# Autodesk Inventor assembly: ASSEMBLY_Visual_inspection_tray
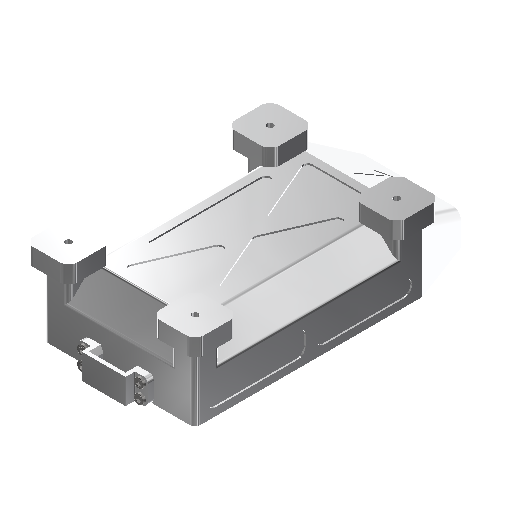
[picture p0: Inventor's stored thumbnail of the model, 512x512]
Saved by Autodesk Inventor 2025 (Build 290162010, 162A)
## iProperties
Created: 2018-09-18
Part Number: ASSEMBLY_Visual_inspection_tray
Document SubType Name: Assembly
Designer: Andrzej
Mass: 50.3843 g
Surface Area: 208.171 cm^2
Volume: 18.5637 cm^3
Density: 2.71413 g/cm^3
Author: Andrzej
## Documents named in this file (5)
- D:\_ANDRZEJ_LACZEWSKI\_OTHER\MECH - My entry for the NASA Lunar Sampling System Design Challenge\MCAD\1_REV1\ASSEMBLY_MAIN_REVA\ASSEMBLY_Visual_inspection_tray.iam
- D:\_ANDRZEJ_LACZEWSKI\_OTHER\MECH - My entry for the NASA Lunar Sampling System Design Challenge\MCAD\1_REV1\ASSEMBLY_MAIN_REVA\CNCM_ALU_Visual_inspection_tray.ipt
- D:\_ANDRZEJ_LACZEWSKI\_OTHER\MECH - My entry for the NASA Lunar Sampling System Design Challenge\MCAD\1_REV1\ASSEMBLY_MAIN_REVA\CNCM_ALU_Visual_inspection_tray_leg_holder.ipt
- D:\_ANDRZEJ_LACZEWSKI\_OTHER\MECH - My entry for the NASA Lunar Sampling System Design Challenge\MCAD\1_REV1\ASSEMBLY_MAIN_REVA\CNCM_ALU_Visial_inspection_tray_bucket_mount.ipt
- D:\_ANDRZEJ_LACZEWSKI\_OTHER\MECH - My entry for the NASA Lunar Sampling System Design Challenge\MCAD\1_REV1\ASSEMBLY_MAIN_REVA\CNCT_STEEL_M1,6x3,5_Screw.ipt
## Components (10 placed, 4 different names)
1. CNCM_ALU_Visual_inspection_tray:1 — Mate:1, Mate:2, Mate:3, Mate:4, Mate:5, Mate:6, Mate:7, Mate:8, Mate:9, Mate:10, Mate:11, Mate:12, Mate:13, Flush:1, Flush:2
2. CNCM_ALU_Visual_inspection_tray_leg_holder:1 — Mate:1, Mate:7, Mate:8
3. CNCM_ALU_Visual_inspection_tray_leg_holder:2 — Mate:2, Mate:9, Mate:10
4. CNCM_ALU_Visual_inspection_tray_leg_holder:3 — Mate:3, Mate:11, Mate:12
5. CNCM_ALU_Visual_inspection_tray_leg_holder:4 — Mate:4, Mate:5, Mate:6
6. CNCM_ALU_Visial_inspection_tray_bucket_mount:1 — Mate:13, Flush:1, Flush:2, Mate:14, Mate:15, Mate:16, Mate:17, Mate:18, Mate:19, Mate:20, Mate:21
7. CNCT_STEEL_M1,6x3,5_Screw:1 — Mate:14, Mate:18
8. CNCT_STEEL_M1,6x3,5_Screw:2 — Mate:15, Mate:19
9. CNCT_STEEL_M1,6x3,5_Screw:3 — Mate:16, Mate:20
10. CNCT_STEEL_M1,6x3,5_Screw:4 — Mate:17, Mate:21
## Relationships (23: Mate 21, Flush 2)
- Mate:1: CNCM_ALU_Visual_inspection_tray:1 ↔ CNCM_ALU_Visual_inspection_tray_leg_holder:1
- Mate:2: CNCM_ALU_Visual_inspection_tray:1 ↔ CNCM_ALU_Visual_inspection_tray_leg_holder:2
- Mate:3: CNCM_ALU_Visual_inspection_tray:1 ↔ CNCM_ALU_Visual_inspection_tray_leg_holder:3
- Mate:4: CNCM_ALU_Visual_inspection_tray:1 ↔ CNCM_ALU_Visual_inspection_tray_leg_holder:4
- Mate:5: CNCM_ALU_Visual_inspection_tray:1 ↔ CNCM_ALU_Visual_inspection_tray_leg_holder:4
- Mate:6: CNCM_ALU_Visual_inspection_tray:1 ↔ CNCM_ALU_Visual_inspection_tray_leg_holder:4
- Mate:7: CNCM_ALU_Visual_inspection_tray:1 ↔ CNCM_ALU_Visual_inspection_tray_leg_holder:1
- Mate:8: CNCM_ALU_Visual_inspection_tray:1 ↔ CNCM_ALU_Visual_inspection_tray_leg_holder:1
- Mate:9: CNCM_ALU_Visual_inspection_tray:1 ↔ CNCM_ALU_Visual_inspection_tray_leg_holder:2
- Mate:10: CNCM_ALU_Visual_inspection_tray:1 ↔ CNCM_ALU_Visual_inspection_tray_leg_holder:2
- Mate:11: CNCM_ALU_Visual_inspection_tray:1 ↔ CNCM_ALU_Visual_inspection_tray_leg_holder:3
- Mate:12: CNCM_ALU_Visual_inspection_tray:1 ↔ CNCM_ALU_Visual_inspection_tray_leg_holder:3
- Mate:13: CNCM_ALU_Visual_inspection_tray:1 ↔ CNCM_ALU_Visial_inspection_tray_bucket_mount:1
- Flush:1: CNCM_ALU_Visual_inspection_tray:1 ↔ CNCM_ALU_Visial_inspection_tray_bucket_mount:1
- Flush:2 (13 mm): CNCM_ALU_Visual_inspection_tray:1 ↔ CNCM_ALU_Visial_inspection_tray_bucket_mount:1
- Mate:14: CNCM_ALU_Visial_inspection_tray_bucket_mount:1 ↔ CNCT_STEEL_M1,6x3,5_Screw:1
- Mate:15: CNCM_ALU_Visial_inspection_tray_bucket_mount:1 ↔ CNCT_STEEL_M1,6x3,5_Screw:2
- Mate:16: CNCM_ALU_Visial_inspection_tray_bucket_mount:1 ↔ CNCT_STEEL_M1,6x3,5_Screw:3
- Mate:17: CNCM_ALU_Visial_inspection_tray_bucket_mount:1 ↔ CNCT_STEEL_M1,6x3,5_Screw:4
- Mate:18: CNCM_ALU_Visial_inspection_tray_bucket_mount:1 ↔ CNCT_STEEL_M1,6x3,5_Screw:1
- Mate:19: CNCM_ALU_Visial_inspection_tray_bucket_mount:1 ↔ CNCT_STEEL_M1,6x3,5_Screw:2
- Mate:20: CNCM_ALU_Visial_inspection_tray_bucket_mount:1 ↔ CNCT_STEEL_M1,6x3,5_Screw:3
- Mate:21: CNCM_ALU_Visial_inspection_tray_bucket_mount:1 ↔ CNCT_STEEL_M1,6x3,5_Screw:4
